# Autodesk Inventor assembly: wheel_assembly
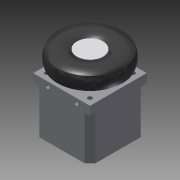
[picture p0: Inventor's stored thumbnail of the model, 180x180]
Saved by Autodesk Inventor 2013 (Build 170138000, 138)
## iProperties
Created: 2013-07-22
Part Number: wheel_assembly
Document SubType Name: Assembly
Designer: dkboone
Author: dkboone
## Documents named in this file (5)
- J:\groups\theresistors\Inventor\wheel_assembly.iam
- J:\groups\theresistors\Inventor\stepper_short.ipt
- J:\groups\theresistors\Inventor\wheel_hub.ipt
- J:\groups\theresistors\Inventor\tire.ipt
- J:\groups\theresistors\Inventor\motor_mount.ipt
## Components (4 placed, 4 different names)
1. stepper_short:1 — Mate:1, Mate:2, Mate:3, Mate:5, Mate:6
2. wheel_hub:1 — Mate:1, Mate:2, Mate:4
3. tire:1 — Mate:3, Mate:4
4. motor_mount:1 — Mate:5, Mate:6
## Relationships (6: Mate 6)
- Mate:1: stepper_short:1 ↔ wheel_hub:1
- Mate:2: stepper_short:1 ↔ wheel_hub:1
- Mate:3: stepper_short:1 ↔ tire:1
- Mate:4 (-5.08 mm): wheel_hub:1 ↔ tire:1
- Mate:5: stepper_short:1 ↔ motor_mount:1
- Mate:6: stepper_short:1 ↔ motor_mount:1
